# Autodesk Inventor assembly: Box
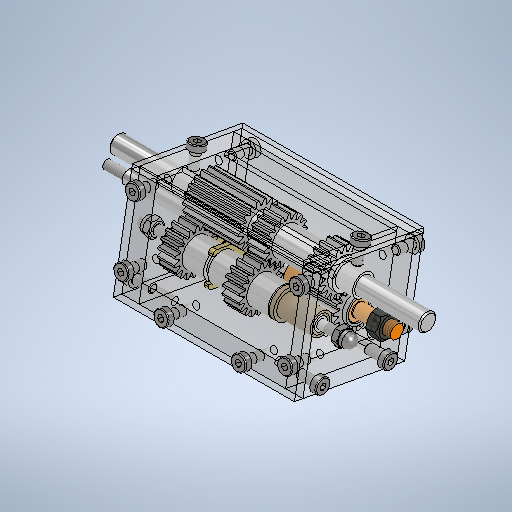
[picture p0: Inventor's stored thumbnail of the model, 512x512]
Saved by Autodesk Inventor 2025 (Build 290162010, 162A)
## iProperties
Created: 2024-07-12
Part Number: Box
Document SubType Name: Assembly
Designer: ffogue
Author: ffogue
## Documents named in this file (19)
- C:\Users\Fabri\Documents\Inventor\GearBox\Box.iam
- C:\Users\Fabri\Documents\Inventor\GearBox\1013.ipt
- C:\Users\Fabri\Documents\Inventor\GearBox\1012.ipt
- C:\Users\Fabri\Documents\Inventor\GearBox\1014.ipt
- C:\Users\Fabri\Documents\Inventor\GearBox\1015.ipt
- C:\Users\Fabri\Documents\Inventor\GearBox\1011.ipt
- C:\Users\Fabri\Documents\Inventor\GearBox\1016.ipt
- C:\Users\Fabri\Documents\Inventor\GearBox\1017ipt.ipt
- C:\Users\Fabri\Documents\Inventor\GearBox\204-Gear.iam
- C:\Users\Fabri\Documents\Inventor\GearBox\1018.ipt
- C:\Users\Fabri\Documents\Inventor\GearBox\202 fitting.ipt
- C:\Users\Fabri\Documents\Inventor\GearBox\202.iam
- C:\Users\Fabri\Documents\Inventor\GearBox\201.iam
- C:\Users\Fabri\Documents\Inventor\GearBox\203.iam
- C:\Users\Fabri\Documents\Inventor\GearBox\102.ipt
- C:\Users\Fabri\Documents\Inventor\GearBox\205 assembly.iam
- C:\Users\Fabri\Documents\Inventor\Content Center Files\R2025\en-US\DIN 1587\DIN 1587 - M4 x 0,7.ipt
- C:\Users\Fabri\Documents\Inventor\Content Center Files\R2025\en-US\ISO 4033(1)\ISO 4033 - M6DIN EN.ipt
- C:\Users\Fabri\Documents\Inventor\Content Center Files\R2025\en-US\DIN 7984\DIN 7984 - M4 x 8.ipt
## Components (38 placed, 18 different names)
1. 1013:1 — Insert:1, Insert:2, Insert:3, Insert:4
2. 1012:1 — Insert:3, Insert:32, Insert:33, Insert:34, Insert:35, Insert:36, Insert:37
3. 1012:2 — Insert:4, Insert:24, Insert:25, Insert:26, Insert:27, Insert:28, Insert:29
4. 1014:1 — Insert:1, Insert:5, Mate:1, Insert:6, Mate:7, Insert:13, Mate:13, Insert:22, Insert:23
5. 1015:1 — Insert:2, Mate:2, Insert:7, Mate:3, Insert:8, Insert:9, Insert:30, Insert:31
6. 1011:1 — Insert:5, Insert:38, Insert:39
7. 1016:1 — Mate:2, Insert:7, Mate:9, Insert:15
8. 1016:2 — Mate:1, Insert:6
9. 1017ipt:1 — Mate:3, Insert:8, Mate:12
10. 204-Gear:1 [sub-assembly] — Mate:5, Insert:9, Insert:10, Insert:17, Tangent:1, Rotation:2, Rotation:3, Insert:18
11. 1018:1 — Mate:5, Insert:10, Mate:11, Insert:19, Insert:20
12. 202:1 [sub-assembly] — Mate:10, Insert:16, Tangent:3, Rotation:3, Rotation:4
13. 201:1 [sub-assembly] — Mate:9, Insert:15, Mate:10, Insert:16, Tangent:1, Rotation:2
14. 203:1 [sub-assembly] — Mate:7, Insert:13, Mate:8, Insert:14, Tangent:3, Rotation:4, Motion
15. 102:1 — Mate:8, Insert:14, Insert:21
16. 202 fitting:1 — Mate:11, Insert:17
17. 205 assembly:1 [sub-assembly] — Mate:12, Insert:18
18. DIN 1587 M4:1 — Insert:19
19. DIN 1587 M4:2 — Insert:20
20. DIN EN 24033 M6:1 — Insert:21
21. DIN 7984 M4 x 8:1 — Insert:31
22. DIN 7984 M4 x 8:2 — Insert:30
23. DIN 7984 M4 x 8:5 — Insert:33
24. DIN 7984 M4 x 8:6 — Insert:37
25. DIN 7984 M4 x 8:7 — Insert:32
26. DIN 7984 M4 x 8:8 — Insert:36
27. DIN 7984 M4 x 8:9 — Insert:35
28. DIN 7984 M4 x 8:10 — Insert:34
29. DIN 7984 M4 x 8:11 — Insert:23
30. DIN 7984 M4 x 8:12 — Mate:13, Insert:22
31. DIN 7984 M4 x 8:13 — Insert:39
32. DIN 7984 M4 x 8:14 — Insert:38
33. DIN 7984 M4 x 8:15 — Insert:29
34. DIN 7984 M4 x 8:16 — Insert:28
35. DIN 7984 M4 x 8:17 — Insert:26
36. DIN 7984 M4 x 8:18 — Insert:25
37. DIN 7984 M4 x 8:19 — Insert:24
38. DIN 7984 M4 x 8:20 — Insert:27
## Relationships (54: Insert 37, Mate 11, RelateRotation 3, Tangent 2, Angle 1)
- Insert:1: 1013:1 ↔ 1014:1
- Insert:2: 1013:1 ↔ 1015:1
- Insert:3: 1013:1 ↔ 1012:1
- Insert:4: 1013:1 ↔ 1012:2
- Insert:5: 1014:1 ↔ 1011:1
- Mate:1: 1014:1 ↔ 1016:2
- Insert:6: 1014:1 ↔ 1016:2
- Mate:2: 1015:1 ↔ 1016:1
- Insert:7: 1015:1 ↔ 1016:1
- Mate:3: 1015:1 ↔ 1017ipt:1
- Insert:8: 1015:1 ↔ 1017ipt:1
- Mate:5: 204-Gear:1 ↔ 1018:1
- Insert:9: 1015:1 ↔ 204-Gear:1
- Insert:10 (-64.5 mm): 204-Gear:1 ↔ 1018:1
- Mate:7: 1014:1 ↔ 203:1
- Insert:13: 1014:1 ↔ 203:1
- Mate:8: 203:1 ↔ 102:1
- Insert:14: 203:1 ↔ 102:1
- Mate:9: 1016:1 ↔ 201:1
- Insert:15: 1016:1 ↔ 201:1
- Mate:10: 202:1 ↔ 201:1
- Insert:16 (2 mm): 202:1 ↔ 201:1
- Mate:11: 1018:1 ↔ 202 fitting:1
- Insert:17: 204-Gear:1 ↔ 202 fitting:1
- Tangent:1: 204-Gear:1 ↔ 201:1
- Tangent:3: 202:1 ↔ 203:1
- Rotation:2 [RelateRotation] (1 ul): 204-Gear:1 ↔ 201:1
- Rotation:3 [RelateRotation] (1 ul): 204-Gear:1 ↔ 202:1
- Rotation:4 [RelateRotation] (1 ul): 202:1 ↔ 203:1
- Mate:12: 1017ipt:1 ↔ 205 assembly:1
- Insert:18: 204-Gear:1 ↔ 205 assembly:1
- Motion [Angle] (720 deg): 203:1
- Insert:19 (-6 mm): 1018:1 ↔ DIN 1587 M4:1
- Insert:20 (-6 mm): 1018:1 ↔ DIN 1587 M4:2
- Insert:21 (-9.5 mm): 102:1 ↔ DIN EN 24033 M6:1
- Mate:13: 1014:1 ↔ DIN 7984 M4 x 8:12
- Insert:22: 1014:1 ↔ DIN 7984 M4 x 8:12
- Insert:23: 1014:1 ↔ DIN 7984 M4 x 8:11
- Insert:24: 1012:2 ↔ DIN 7984 M4 x 8:19
- Insert:25: 1012:2 ↔ DIN 7984 M4 x 8:18
- Insert:26: 1012:2 ↔ DIN 7984 M4 x 8:17
- Insert:27: 1012:2 ↔ DIN 7984 M4 x 8:20
- Insert:28: 1012:2 ↔ DIN 7984 M4 x 8:16
- Insert:29: 1012:2 ↔ DIN 7984 M4 x 8:15
- Insert:30: 1015:1 ↔ DIN 7984 M4 x 8:2
- Insert:31: 1015:1 ↔ DIN 7984 M4 x 8:1
- Insert:32: 1012:1 ↔ DIN 7984 M4 x 8:7
- Insert:33: 1012:1 ↔ DIN 7984 M4 x 8:5
- Insert:34: 1012:1 ↔ DIN 7984 M4 x 8:10
- Insert:35: 1012:1 ↔ DIN 7984 M4 x 8:9
- Insert:36: 1012:1 ↔ DIN 7984 M4 x 8:8
- Insert:37: 1012:1 ↔ DIN 7984 M4 x 8:6
- Insert:38: 1011:1 ↔ DIN 7984 M4 x 8:14
- Insert:39: 1011:1 ↔ DIN 7984 M4 x 8:13
